# Autodesk Inventor assembly: Turret Base
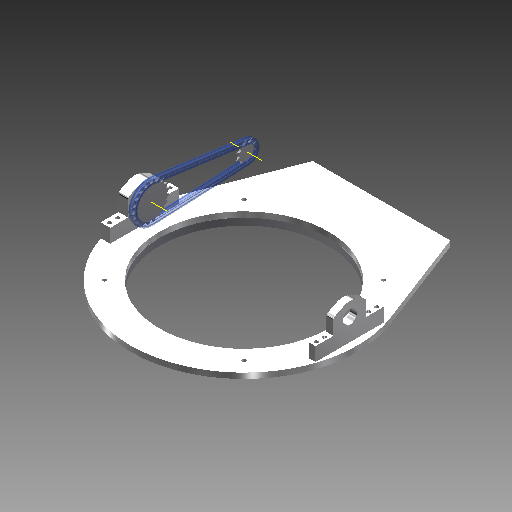
[picture p0: Inventor's stored thumbnail of the model, 512x512]
Saved by Autodesk Inventor 2019.4 (Build 234330000, 330)
## iProperties
Created: 2020-01-06
Part Number: Turret Base
Document SubType Name: Assembly
Designer: admin
Author: admin
## Documents named in this file (7)
- C:\Users\Mark\Desktop\7738 Helion Engineering\7738-2020\Turret\Turret Base.iam
- C:\Users\Mark\Desktop\7738 Helion Engineering\7738-2020\Turret\Slewing Bearing.ipt
- C:\Users\Mark\Desktop\7738 Helion Engineering\7738-2020\Turret\Turret Base\Design Accelerator\Chain Drive1.iam
- C:\Users\Mark\Desktop\7738 Helion Engineering\7738-2020\Turret\Turret Base Plate.ipt
- C:\Users\Mark\Desktop\7738 Helion Engineering\7738-2020\Turret\Bearing Block Dual.ipt
- C:\Users\Mark\Desktop\7738 Helion Engineering\7738-2020\CAD\Gearbox\F6804.ipt
- C:\Users\Mark\Desktop\7738 Helion Engineering\7738-2020\Turret\Axle Block.ipt
## Components (7 placed, 6 different names)
1. Slewing Bearing:1 — Mate:1, Mate:2, Mate:5, Mate:6, Mate:7
2. Chain Drive:1 [sub-assembly]
3. Turret Base Plate:1 — Mate:5, Mate:6, Mate:7, Mate:15, Angle:2, Mate:18, Mate:20, Mate:21, Mate:22, Mate:23
4. Bearing Block Dual:1 — Mate:11, Mate:12, Mate:13, Mate:14, Mate:15, Mate:22, Mate:23
5. F6804:1 — Mate:11, Mate:14
6. F6804:2 — Mate:12, Mate:13
7. Axle Block:1 — Mate:18, Mate:20, Mate:21
## Relationships (16: Mate 15, Angle 1)
- Mate:1: Slewing Bearing:1
- Mate:2: Slewing Bearing:1
- Mate:5: Slewing Bearing:1 ↔ Turret Base Plate:1
- Mate:6: Slewing Bearing:1 ↔ Turret Base Plate:1
- Mate:7: Slewing Bearing:1 ↔ Turret Base Plate:1
- Mate:11: Bearing Block Dual:1 ↔ F6804:1
- Mate:12: Bearing Block Dual:1 ↔ F6804:2
- Mate:13 (0.2 mm): Bearing Block Dual:1 ↔ F6804:2
- Mate:14 (0.2 mm): Bearing Block Dual:1 ↔ F6804:1
- Mate:15: Turret Base Plate:1 ↔ Bearing Block Dual:1
- Angle:2 (180 deg): Turret Base Plate:1
- Mate:18: Turret Base Plate:1 ↔ Axle Block:1
- Mate:20: Turret Base Plate:1 ↔ Axle Block:1
- Mate:21: Turret Base Plate:1 ↔ Axle Block:1
- Mate:22: Turret Base Plate:1 ↔ Bearing Block Dual:1
- Mate:23: Turret Base Plate:1 ↔ Bearing Block Dual:1
